# Autodesk Inventor assembly: Сборка1
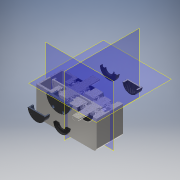
[picture p0: Inventor's stored thumbnail of the model, 180x180]
Saved by Autodesk Inventor 2016 (Build 200138000, 138)
## iProperties
Created: 2021-04-23
Part Number: Сборка1
Material: Типовые
Document SubType Name: Assembly
Designer: Лол
Author: Лол
## Documents named in this file (23)
- C:\Users\Лол\Documents\Inventor\course_work\Сборка1.iam
- C:\Users\Лол\Documents\Inventor\course_work\корпус01.ipt
- C:\Users\Лол\Documents\Inventor\course_work\Подшипник.ipt
- C:\Users\Лол\Documents\Inventor\course_work\Подшипник\Подшипник-02.ipt
- C:\Users\Лол\Documents\Inventor\course_work\Small.ipt
- C:\Users\Лол\Documents\Inventor\course_work\big.ipt
- C:\Users\Лол\Documents\Inventor\course_work\Wheel.ipt
- C:\Users\Лол\Documents\Inventor\course_work\Кольцо A30 ГОСТ 13942-86.ipt
- C:\Users\Лол\Documents\Inventor\course_work\Кольцо A35 ГОСТ 13942-86.ipt
- C:\Users\Лол\Documents\Inventor\course_work\Гайка M33x1.5 6H ГОСТ 6393-73.ipt
- C:\Users\Лол\Documents\Inventor\course_work\Гайка M30x1.5 6H ГОСТ 6393-73.ipt
- C:\Users\Лол\Documents\Inventor\course_work\Корпус02.ipt
- C:\Users\Лол\Documents\Inventor\course_work\Подшипник\Подшипник-01.ipt
- C:\Users\Лол\Documents\Inventor\course_work\Манжет 1-30x72x10 ГОСТ 8752-79.ipt
- C:\Users\Лол\Documents\Inventor\course_work\Манжет 1-28x62x10 ГОСТ 8752-79.ipt
- C:\Users\Лол\Documents\Inventor\course_work\Крышка маленькая.ipt
- C:\Users\Лол\Documents\Inventor\course_work\Крышка большая.ipt
- C:\Users\Лол\Documents\Inventor\course_work\корпус01_ЗЕРКАЛО.ipt
- C:\Users\Лол\Documents\Inventor\course_work\AS 1420 - 1973 - M10 x 75.ipt
- C:\Users\Лол\Documents\Inventor\course_work\ISO 2340 - A - 6 x 40ISO.ipt
- C:\Users\Лол\Documents\Inventor\course_work\Крышка большая_72.ipt
- C:\Users\Лол\Documents\Inventor\course_work\Крышка маленькая_62.ipt
- C:\Users\Лол\Documents\Inventor\course_work\КОДЬЦО 062-066-25 гост 9833.ipt
## Components (29 placed, 21 different names)
1. корпус01:1 — Совмещение:1, Совмещение:2, Заподлицо:1, Совмещение:20, Совмещение:21, Совмещение:30, Совмещение:31, Совмещение:32, Совмещение:33, Совмещение:34, Совмещение:41, Совмещение:46, Совмещение:64, Совмещение:65, Совмещение:66, Совмещение:67, Совмещение:68, Совмещение:69, Совмещение:70, Совмещение:71, Совмещение:72, Угол:1, Совмещение:79, Заподлицо:5, Совмещение:83, Совмещение:84
2. big:1 — Совмещение:9, Совмещение:10, Совмещение:15, Совмещение:16, Совмещение:17, Совмещение:35, Совмещение:47, Совмещение:57
3. Small:1 — Совмещение:13, Совмещение:14, Совмещение:37, Совмещение:38, Совмещение:42
4. Wheel:1 — Совмещение:9, Совмещение:10, Совмещение:36
5. Кольцо A30 ГОСТ 13942-86:1 — Совмещение:13, Совмещение:14
6. Кольцо A35 ГОСТ 13942-86:1 — Совмещение:15, Совмещение:16
7. Гайка M33x1.5 6H ГОСТ 6393-73:1 — Совмещение:17, Совмещение:39, Совмещение:40
8. Корпус02:1 — Совмещение:20, Совмещение:21, Совмещение:30, Совмеще1ние:58, Совмещение:74, Заподлицо:2, Совмещение:75, Заподлицо:3
9. Подшипник-01:1 — Совмещение:31, Совмещение:34, Совмещение:37, Совмещение:38, Совмещение:45
10. Подшипник-02:2 — Совмещение:32, Совмещение:33, Совмещение:35, Совмещение:36, Совмещение:39
11. Манжет 1-30x72x10 ГОСТ 8752-79:2 — Совмещение:40, Совмещение:41
12. Гайка M30x1.5 6H ГОСТ 6393-73:1 — Совмещение:42, Совмещение:43, Совмещение:44, Совмещение:55
13. Манжет 1-28x62x10 ГОСТ 8752-79:4 — Совмещение:43, Совмещение:44
14. Крышка маленькая:1 — Совмещение:45, Совмещение:46
15. Крышка большая:2 — Совмещение:47, Совмещение:54
16. Подшипник-01:3 — Совмещение:55, Совмещение:61, Совмещение:62
17. Подшипник-02:4 — Совмещение:54, Совмещение:57, Совмещение:63
18. корпус01_ЗЕРКАЛО:1 — Совмеще1ние:58, Совмещение:59, Совмещение:60, Совмещение:61, Совмещение:62, Совмещение:63, Совмещение:76, Совмещение:77, Совмещение:78, Заподлицо:4, Совмещение:80, Совмещение:81
19. AS 1420 - 1973 - M10 x 75:1 — Совмещение:65, Совмещение:70
20. AS 1420 - 1973 - M10 x 75:2 — Совмещение:64, Совмещение:69
21. AS 1420 - 1973 - M10 x 75:3 — Совмещение:67, Совмещение:68
22. AS 1420 - 1973 - M10 x 75:4 — Совмещение:66, Совмещение:71
23. ISO 2340 - A - 6 x 40ISO:2 — Совмещение:74, Заподлицо:2, Совмещение:77
24. ISO 2340 - A - 6 x 40ISO:3 — Совмещение:75, Заподлицо:3, Совмещение:76
25. Манжет 1-28x62x10 ГОСТ 8752-79:5 — Совмещение:78, Заподлицо:4
26. Манжет 1-30x72x10 ГОСТ 8752-79:3 — Совмещение:79, Заподлицо:5
27. Крышка большая_72:1 — Совмещение:80, Совмещение:81, Совмещение:82
28. Крышка маленькая_62:5 — Совмещение:83, Совмещение:84, Угол:2, Совмещение:85, Касательность:1
29. КОДЬЦО 062-066-25 гост 9833:1 — Совмещение:85, Касательность:1
## Relationships (68: Mate 60, Flush 5, Angle 2, Tangent 1)
- Совмещение:1 [Mate]: корпус01:1
- Совмещение:2 [Mate]: корпус01:1
- Заподлицо:1 [Flush]: корпус01:1
- Совмещение:9 [Mate]: big:1 ↔ Wheel:1
- Совмещение:10 [Mate]: big:1 ↔ Wheel:1
- Совмещение:13 [Mate]: Small:1 ↔ Кольцо A30 ГОСТ 13942-86:1
- Совмещение:14 [Mate]: Small:1 ↔ Кольцо A30 ГОСТ 13942-86:1
- Совмещение:15 [Mate]: big:1 ↔ Кольцо A35 ГОСТ 13942-86:1
- Совмещение:16 [Mate]: big:1 ↔ Кольцо A35 ГОСТ 13942-86:1
- Совмещение:17 [Mate]: big:1 ↔ Гайка M33x1.5 6H ГОСТ 6393-73:1
- Совмещение:20 [Mate]: корпус01:1 ↔ Корпус02:1
- Совмещение:21 [Mate]: корпус01:1 ↔ Корпус02:1
- Совмещение:30 [Mate]: корпус01:1 ↔ Корпус02:1
- Совмещение:31 [Mate]: корпус01:1 ↔ Подшипник-01:1
- Совмещение:32 [Mate]: корпус01:1 ↔ Подшипник-02:2
- Совмещение:33 [Mate]: корпус01:1 ↔ Подшипник-02:2
- Совмещение:34 [Mate]: корпус01:1 ↔ Подшипник-01:1
- Совмещение:35 [Mate]: big:1 ↔ Подшипник-02:2
- Совмещение:36 [Mate] (10 mm): Wheel:1 ↔ Подшипник-02:2
- Совмещение:37 [Mate]: Small:1 ↔ Подшипник-01:1
- Совмещение:38 [Mate] (9 mm): Small:1 ↔ Подшипник-01:1
- Совмещение:39 [Mate]: Гайка M33x1.5 6H ГОСТ 6393-73:1 ↔ Подшипник-02:2
- Совмещение:40 [Mate] (100 mm): Гайка M33x1.5 6H ГОСТ 6393-73:1 ↔ Манжет 1-30x72x10 ГОСТ 8752-79:2
- Совмещение:41 [Mate]: корпус01:1 ↔ Манжет 1-30x72x10 ГОСТ 8752-79:2
- Совмещение:42 [Mate]: Small:1 ↔ Гайка M30x1.5 6H ГОСТ 6393-73:1
- Совмещение:43 [Mate] (100 mm): Гайка M30x1.5 6H ГОСТ 6393-73:1 ↔ Манжет 1-28x62x10 ГОСТ 8752-79:4
- Совмещение:44 [Mate]: Гайка M30x1.5 6H ГОСТ 6393-73:1 ↔ Манжет 1-28x62x10 ГОСТ 8752-79:4
- Совмещение:45 [Mate] (100 mm): Подшипник-01:1 ↔ Крышка маленькая:1
- Совмещение:46 [Mate]: корпус01:1 ↔ Крышка маленькая:1
- Совмещение:47 [Mate]: big:1 ↔ Крышка большая:2
- Совмещение:54 [Mate] (100 mm): Крышка большая:2 ↔ Подшипник-02:4
- Совмещение:55 [Mate]: Гайка M30x1.5 6H ГОСТ 6393-73:1 ↔ Подшипник-01:3
- Совмещение:57 [Mate]: big:1 ↔ Подшипник-02:4
- Совмеще1ние:58 [Mate]: Корпус02:1 ↔ корпус01_ЗЕРКАЛО:1
- Совмещение:59 [Mate]: корпус01_ЗЕРКАЛО:1
- Совмещение:60 [Mate]: корпус01_ЗЕРКАЛО:1
- Совмещение:61 [Mate]: Подшипник-01:3 ↔ корпус01_ЗЕРКАЛО:1
- Совмещение:62 [Mate]: Подшипник-01:3 ↔ корпус01_ЗЕРКАЛО:1
- Совмещение:63 [Mate]: Подшипник-02:4 ↔ корпус01_ЗЕРКАЛО:1
- Совмещение:64 [Mate]: корпус01:1 ↔ AS 1420 - 1973 - M10 x 75:2
- Совмещение:65 [Mate]: корпус01:1 ↔ AS 1420 - 1973 - M10 x 75:1
- Совмещение:66 [Mate]: корпус01:1 ↔ AS 1420 - 1973 - M10 x 75:4
- Совмещение:67 [Mate]: корпус01:1 ↔ AS 1420 - 1973 - M10 x 75:3
- Совмещение:68 [Mate]: корпус01:1 ↔ AS 1420 - 1973 - M10 x 75:3
- Совмещение:69 [Mate]: корпус01:1 ↔ AS 1420 - 1973 - M10 x 75:2
- Совмещение:70 [Mate]: корпус01:1 ↔ AS 1420 - 1973 - M10 x 75:1
- Совмещение:71 [Mate]: корпус01:1 ↔ AS 1420 - 1973 - M10 x 75:4
- Совмещение:72 [Mate]: корпус01:1
- Совмещение:73 [Mate]
- Угол:1 [Angle] (0 deg): корпус01:1
- Совмещение:74 [Mate]: Корпус02:1 ↔ ISO 2340 - A - 6 x 40ISO:2
- Заподлицо:2 [Flush] (7.5 mm): Корпус02:1 ↔ ISO 2340 - A - 6 x 40ISO:2
- Совмещение:75 [Mate]: Корпус02:1 ↔ ISO 2340 - A - 6 x 40ISO:3
- Заподлицо:3 [Flush] (-7.5 mm): Корпус02:1 ↔ ISO 2340 - A - 6 x 40ISO:3
- Совмещение:76 [Mate]: корпус01_ЗЕРКАЛО:1 ↔ ISO 2340 - A - 6 x 40ISO:3
- Совмещение:77 [Mate]: корпус01_ЗЕРКАЛО:1 ↔ ISO 2340 - A - 6 x 40ISO:2
- Совмещение:78 [Mate]: корпус01_ЗЕРКАЛО:1 ↔ Манжет 1-28x62x10 ГОСТ 8752-79:5
- Заподлицо:4 [Flush]: корпус01_ЗЕРКАЛО:1 ↔ Манжет 1-28x62x10 ГОСТ 8752-79:5
- Совмещение:79 [Mate]: корпус01:1 ↔ Манжет 1-30x72x10 ГОСТ 8752-79:3
- Заподлицо:5 [Flush]: корпус01:1 ↔ Манжет 1-30x72x10 ГОСТ 8752-79:3
- Совмещение:80 [Mate]: корпус01_ЗЕРКАЛО:1 ↔ Крышка большая_72:1
- Совмещение:81 [Mate]: корпус01_ЗЕРКАЛО:1 ↔ Крышка большая_72:1
- Совмещение:82 [Mate]: Крышка большая_72:1
- Совмещение:83 [Mate]: корпус01:1 ↔ Крышка маленькая_62:5
- Совмещение:84 [Mate]: корпус01:1 ↔ Крышка маленькая_62:5
- Угол:2 [Angle] (0 deg): Крышка маленькая_62:5
- Совмещение:85 [Mate]: Крышка маленькая_62:5 ↔ КОДЬЦО 062-066-25 гост 9833:1
- Касательность:1 [Tangent]: Крышка маленькая_62:5 ↔ КОДЬЦО 062-066-25 гост 9833:1
